# Autodesk Inventor assembly: HbSocketU02
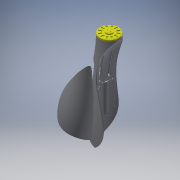
[picture p0: Inventor's stored thumbnail of the model, 180x180]
Saved by Autodesk Inventor 2017 (Build 210142000, 142)
## iProperties
Created: 2015-02-09
Part Number: HbSocketU02
Document SubType Name: Assembly
Designer: Yamaura
Author: Yamaura
## Documents named in this file (12)
- D:\OneDrive\CAD\MAJ\hackberry\HACKberry-hardware\3D_69%inlength\Inventor\HbSocketU02ForChild\HbSocketU02ForChild.iam
- D:\OneDrive\CAD\MAJ\hackberry\HACKberry-hardware\3D_69%inlength\Inventor\HbSocketU02ForChild\HbBatteryDoor03.ipt
- D:\OneDrive\CAD\MAJ\hackberry\HACKberry-hardware\3D_69%inlength\Inventor\HbSocketU02ForChild\HbBatteryDoorKnob03.ipt
- D:\OneDrive\CAD\MAJ\hackberry\HACKberry-hardware\3D_69%inlength\Inventor\HbSocketU02ForChild\HbBatteryHingeA03.ipt
- D:\OneDrive\CAD\MAJ\hackberry\HACKberry-hardware\3D_69%inlength\Inventor\HbSocketU02ForChild\HbBatteryHingeB03.ipt
- D:\OneDrive\CAD\MAJ\hackberry\HACKberry-hardware\3D_69%inlength\Inventor\HbSocketU02ForChild\HbBatteryHingeC03.ipt
- D:\OneDrive\CAD\MAJ\hackberry\HACKberry-hardware\3D_69%inlength\Inventor\HbSocketU02ForChild\HbBatteryDoorLever03.ipt
- D:\OneDrive\CAD\MAJ\hackberry\HACKberry-hardware\3D_69%inlength\Inventor\HbSocketU02ForChild\HbMainFrameA01.ipt
- D:\OneDrive\CAD\MAJ\hackberry\HACKberry-hardware\3D_69%inlength\Inventor\HbSocketU02ForChild\HbMainFrameB01.ipt
- D:\OneDrive\CAD\MAJ\hackberry\HACKberry-hardware\3D_69%inlength\Inventor\HbSocketU02ForChild\TS 0.4-3.2-14.ipt
- D:\OneDrive\CAD\MAJ\hackberry\HACKberry-hardware\3D_69%inlength\Inventor\HbSocketU02ForChild\HbWristLockPlate01.ipt
- D:\OneDrive\CAD\MAJ\hackberry\HACKberry-hardware\3D_69%inlength\Inventor\HbSocketU02ForChild\battery_R6.ipt
## Components (15 placed, 11 different names)
1. TS 0.4-3.2-14:1
2. HbBatteryHingeC03:1 — 挿入:6, 挿入:7
3. HbBatteryHingeB03:1 — 挿入:8, 挿入:9
4. HbBatteryHingeA03:1 — 挿入:10, 挿入:11
5. HbBatteryDoor03:1 — 挿入:6, 挿入:7, 挿入:8, 挿入:9, 挿入:10, 挿入:11, 挿入:12
6. HbMainFrameA01:1 — 挿入:1, 挿入:2, メイト:1, メイト:2, 挿入:4, 挿入:5
7. HbBatteryDoorKnob03:3 — メイト:1, メイト:2, 挿入:3
8. HbMainFrameB01:1 — 挿入:4, 挿入:5, 挿入:12
9. HbWristLockPlate01:1 — 挿入:1, 挿入:2
10. battery_R6:1
11. battery_R6:2
12. HbBatteryDoorKnob03:1
13. HbBatteryDoorKnob03:2
14. HbBatteryDoorLever03:1
15. HbBatteryDoorLever03:2 — 挿入:3
## Component patterns: (2 elements, first: HbBatteryDoorKnob03:1), (2 elements, first: HbBatteryDoorLever03:1)
## Relationships (14: Insert 12, Mate 2)
- 挿入:1 [Insert]: HbMainFrameA01:1 ↔ HbWristLockPlate01:1
- 挿入:2 [Insert]: HbMainFrameA01:1 ↔ HbWristLockPlate01:1
- メイト:1 [Mate]: HbMainFrameA01:1 ↔ HbBatteryDoorKnob03:3
- メイト:2 [Mate]: HbMainFrameA01:1 ↔ HbBatteryDoorKnob03:3
- 挿入:3 [Insert]: HbBatteryDoorKnob03:3 ↔ HbBatteryDoorLever03:2
- 挿入:4 [Insert]: HbMainFrameA01:1 ↔ HbMainFrameB01:1
- 挿入:5 [Insert]: HbMainFrameA01:1 ↔ HbMainFrameB01:1
- 挿入:6 [Insert]: HbBatteryHingeC03:1 ↔ HbBatteryDoor03:1
- 挿入:7 [Insert]: HbBatteryHingeC03:1 ↔ HbBatteryDoor03:1
- 挿入:8 [Insert]: HbBatteryHingeB03:1 ↔ HbBatteryDoor03:1
- 挿入:9 [Insert]: HbBatteryHingeB03:1 ↔ HbBatteryDoor03:1
- 挿入:10 [Insert]: HbBatteryHingeA03:1 ↔ HbBatteryDoor03:1
- 挿入:11 [Insert]: HbBatteryHingeA03:1 ↔ HbBatteryDoor03:1
- 挿入:12 [Insert]: HbBatteryDoor03:1 ↔ HbMainFrameB01:1
